# Autodesk Inventor assembly: !structure_half
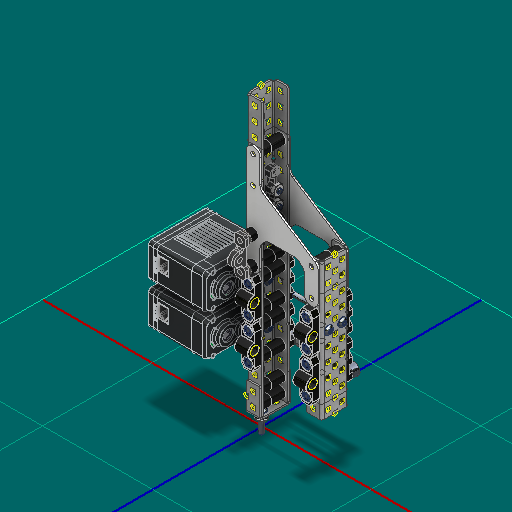
[picture p0: Inventor's stored thumbnail of the model, 512x512]
Saved by Autodesk Inventor 2025 (Build 290162000, 162)
## iProperties
Created: 2024-08-20
Part Number: !structure_half
Document SubType Name: Assembly
Designer: averey
Author: averey
## Documents named in this file (21)
- C:\Users\avere\vex_robotics_high_stakes\hardware\cad\ATLAS\tower\structure\!structure_half.iam
- C:\Users\avere\vex_robotics_high_stakes\hardware\cad\ATLAS\tower\structure\structure_channel.iam
- C:\Users\avere\vex_robotics_high_stakes\hardware\cad\ATLAS\tower\structure\intake_gearbox_outer.iam
- C:\Users\avere\vex_robotics_high_stakes\hardware\cad\custom_parts\modified_parts\Bearing Flat Low Profile 2-Hole.ipt
- C:\Users\avere\vex_robotics_high_stakes\hardware\cad\VEX-CAD-Inventor\Structure\Hardware\Screw Steel - Star\SScrew Star Smooth 1.750.ipt
- C:\Users\avere\vex_robotics_high_stakes\hardware\cad\VEX-CAD-Inventor\Structure\Hardware\Screw Steel - Star.ipt
- C:\Users\avere\vex_robotics_high_stakes\hardware\cad\VEX-CAD-Inventor\Structure\Hardware\Screw Shoulder Robosource\SScrew Shoulder Smooth .500 x .04.ipt
- C:\Users\avere\vex_robotics_high_stakes\hardware\cad\VEX-CAD-Inventor\Structure\Hardware\Screw Shoulder Robosource.ipt
- C:\Users\avere\vex_robotics_high_stakes\hardware\cad\VEX-CAD-Inventor\Structure\Hardware\Nut Thin Nylock.ipt
- C:\Users\avere\vex_robotics_high_stakes\hardware\cad\ATLAS\tower\gusset.ipt
- C:\Users\avere\vex_robotics_high_stakes\hardware\cad\VEX-CAD-Inventor\Motion\Shaft LS\LS Pillow Bearing Block.ipt
- C:\Users\avere\vex_robotics_high_stakes\hardware\cad\VEX-CAD-Inventor\Motion\Spacers\Spacer Nylon .375 OD\NSpacer .375 OD x .250.ipt
- C:\Users\avere\vex_robotics_high_stakes\hardware\cad\VEX-CAD-Inventor\Motion\Spacers\Spacer Nylon .375 OD.ipt
- C:\Users\avere\vex_robotics_high_stakes\hardware\cad\VEX-CAD-Inventor\Motion\Spacers\Washer Steel\SWasher .375 OD x .015625.ipt
- C:\Users\avere\vex_robotics_high_stakes\hardware\cad\VEX-CAD-Inventor\Motion\Spacers\Washer Steel.ipt
- C:\Users\avere\vex_robotics_high_stakes\hardware\cad\VEX-CAD-Inventor\Motion\Spacers\Washer Steel\SWasher .375 OD x .031250.ipt
- C:\Users\avere\vex_robotics_high_stakes\hardware\cad\VEX-CAD-Inventor\Motion\Spacers\Washer Steel\SWasher .375 OD x .062500.ipt
- C:\Users\avere\vex_robotics_high_stakes\hardware\cad\VEX-CAD-Inventor\Motion\Shaft LS\Shaft Collar ipts\Shaft Collar No Screw.ipt
- C:\Users\avere\vex_robotics_high_stakes\hardware\cad\VEX-CAD-Inventor\Motion\Spacers\Spacer Nylon .375 OD\NSpacer .375 OD x .125.ipt
- C:\Users\avere\vex_robotics_high_stakes\hardware\cad\VEX-CAD-Inventor\Structure\Standoff\Standoff 1.50.ipt
- C:\Users\avere\vex_robotics_high_stakes\hardware\cad\VEX-CAD-Inventor\Structure\Standoff.ipt
## Components (22 placed, 15 different names)
1. structure_channel:1 [sub-assembly] — Mate:8
2. intake_gearbox_outer:1 [sub-assembly] — Angle:2
3. Bearing Flat Low Profile 2-Hole:1
4. SScrew Star Smooth 1.750:1
5. SScrew Shoulder Smooth .500 x .04:1
6. Nut Thin Nylock:1
7. gusset:1
8. gusset:2 — Angle:1
9. LS Pillow Bearing Block:1
10. NSpacer .375 OD x .250:1
11. SWasher .375 OD x .015625:1
12. SWasher .375 OD x .031250:2
13. SWasher .375 OD x .062500:3
14. NSpacer .375 OD x .250:2
15. SWasher .375 OD x .015625:4
16. SWasher .375 OD x .031250:5
17. SWasher .375 OD x .062500:6
18. Shaft Collar No Screw:1
19. Shaft Collar No Screw:2
20. NSpacer .375 OD x .125:3
21. SWasher .375 OD x .062500:7
22. Standoff 1.50:1
## Relationships (31: Insert 21, Mate 8, Angle 2)
- [Mate]: structure_channel:1 ↔ intake_gearbox_outer:1
- [Insert]: intake_gearbox_outer:1 ↔ Bearing Flat Low Profile 2-Hole:1
- [Mate]: intake_gearbox_outer:1 ↔ Bearing Flat Low Profile 2-Hole:1
- [Insert]: intake_gearbox_outer:1 ↔ SScrew Star Smooth 1.750:1
- [Insert] (1.27 mm): Bearing Flat Low Profile 2-Hole:1 ↔ Nut Thin Nylock:1
- [Insert]: intake_gearbox_outer:1 ↔ SScrew Shoulder Smooth .500 x .04:1
- [Insert] (25.4 mm): gusset:1 ↔ gusset:2
- [Mate]: gusset:1 ↔ gusset:2
- [Insert]: structure_channel:1 ↔ gusset:2
- [Mate]: structure_channel:1 ↔ gusset:2
- [Insert]: NSpacer .375 OD x .250:1 ↔ SWasher .375 OD x .062500:3
- [Insert]: SWasher .375 OD x .031250:2 ↔ SWasher .375 OD x .062500:3
- [Insert]: SWasher .375 OD x .015625:1 ↔ SWasher .375 OD x .031250:2
- [Insert]: NSpacer .375 OD x .250:2 ↔ SWasher .375 OD x .062500:6
- [Insert]: SWasher .375 OD x .031250:5 ↔ SWasher .375 OD x .062500:6
- [Insert]: SWasher .375 OD x .015625:4 ↔ SWasher .375 OD x .031250:5
- [Insert]: LS Pillow Bearing Block:1 ↔ SWasher .375 OD x .015625:4
- [Insert]: LS Pillow Bearing Block:1 ↔ SWasher .375 OD x .015625:1
- [Insert]: gusset:2 ↔ NSpacer .375 OD x .250:1
- [Mate]: gusset:2 ↔ NSpacer .375 OD x .250:2
- [Insert]: intake_gearbox_outer:1 ↔ gusset:2
- [Mate]: intake_gearbox_outer:1 ↔ gusset:2
- [Insert]: intake_gearbox_outer:1 ↔ Shaft Collar No Screw:1
- [Insert]: structure_channel:1 ↔ Shaft Collar No Screw:2
- [Mate]: Shaft Collar No Screw:1 ↔ Shaft Collar No Screw:2
- [Insert]: NSpacer .375 OD x .125:3 ↔ SWasher .375 OD x .062500:7
- [Insert]: SWasher .375 OD x .062500:7 ↔ Standoff 1.50:1
- [Insert]: Shaft Collar No Screw:1 ↔ NSpacer .375 OD x .125:3
- Mate:8: structure_channel:1
- Angle:1 (0 deg): gusset:2
- Angle:2 (0 deg): intake_gearbox_outer:1
## Named parameters: d116_d113 = 0 mm, d117_d114 = 0 mm, d118_d115 = 0 mm
